# Autodesk Inventor assembly: Cylinder Assembly
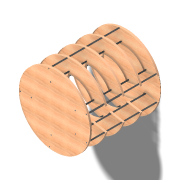
[picture p0: Inventor's stored thumbnail of the model, 180x180]
Saved by Autodesk Inventor 2021 (Build 250183000, 183)
## iProperties
Created: 2020-11-06
Part Number: Cylinder Assembly
Document SubType Name: Assembly
Designer: Dan Wikman
Author: Dan Wikman
## Documents named in this file (12)
- C:\Users\Dan Wikman\OneDrive\University Life\2020, Semester 1\METR4900 Honours Thesis\Cylindrical Mock Up\Cylinder Assembly.iam
- C:\Users\Dan Wikman\OneDrive\University Life\2020, Semester 1\METR4900 Honours Thesis\Cylindrical Mock Up\Rod.ipt
- C:\Users\Dan Wikman\OneDrive\University Life\2020, Semester 1\METR4900 Honours Thesis\Cylindrical Mock Up\Shelf.ipt
- C:\Users\Dan Wikman\OneDrive\University Life\2020, Semester 1\METR4900 Honours Thesis\Cylindrical Mock Up\TopandBase.ipt
- C:\Users\Dan Wikman\OneDrive\University Life\2020, Semester 1\METR4900 Honours Thesis\Cylindrical Mock Up\Shelf Edge Banding.ipt
- C:\Users\Dan Wikman\OneDrive\University Life\2020, Semester 1\METR4900 Honours Thesis\Cylindrical Mock Up\Roof Banding.ipt
- C:\Users\Dan Wikman\OneDrive\University Life\2020, Semester 1\METR4900 Honours Thesis\Cylindrical Mock Up\Cylinder Assembly\AIP\FEA\df0owmtmo.fins
- C:\Users\Dan Wikman\OneDrive\University Life\2020, Semester 1\METR4900 Honours Thesis\Cylindrical Mock Up\Cylinder Assembly\AIP\FEA\df0owmtmo.fsat
- C:\Users\Dan Wikman\OneDrive\University Life\2020, Semester 1\METR4900 Honours Thesis\Cylindrical Mock Up\Cylinder Assembly\AIP\FEA\df0owmtmo.ftes
- C:\Users\Dan Wikman\OneDrive\University Life\2020, Semester 1\METR4900 Honours Thesis\Cylindrical Mock Up\Cylinder Assembly\AIP\FEA\df0owmtmo.fwiz
- C:\Users\Dan Wikman\OneDrive\University Life\2020, Semester 1\METR4900 Honours Thesis\Cylindrical Mock Up\Cylinder Assembly\AIP\FEA\df0owmtq8.fmsh
- C:\Users\Dan Wikman\OneDrive\University Life\2020, Semester 1\METR4900 Honours Thesis\Cylindrical Mock Up\Cylinder Assembly\AIP\FEA\df0owmtq9.fres
## Components (20 placed, 5 different names)
1. Rod:1 — Mate:3, Flush:1, Mate:4, Flush:2
2. Shelf:1 — Mate:1, Mate:2, Mate:3, Mate:26, Mate:27, Flush:7
3. TopandBase:1 — Mate:1, Mate:2, Flush:1, Mate:5, Mate:6, Mate:7, Mate:8, Mate:9, Mate:10, Mate:11, Mate:12, Mate:13, Mate:14, Mate:28, Mate:38, Mate:45, Flush:11
4. TopandBase:2 — Mate:4, Mate:5, Flush:2, Mate:43, Mate:46
5. Rod:2 — Mate:8
6. Rod:3 — Mate:9
7. Rod:4 — Mate:10
8. Rod:5 — Mate:11
9. Rod:6 — Mate:12
10. Rod:7 — Mate:13, Mate:33, Mate:35
11. Rod:8 — Mate:14, Mate:34, Mate:36
12. Rod:9 — Mate:7
13. Rod:10 — Mate:6
14. Shelf Edge Banding:1 — Mate:26, Mate:27, Flush:7, Mate:28
15. Shelf:2 — Mate:33, Mate:34
16. Shelf Edge Banding:2 — Mate:38
17. Shelf:3 — Mate:35, Mate:36
18. Shelf Edge Banding:3 — Flush:10, Mate:44, Mate:46
19. Shelf Edge Banding:4 — Mate:43, Flush:10, Mate:44
20. Roof Banding:1 — Mate:45, Flush:11
## Relationships (37: Mate 30, Flush 7)
- Mate:1: Shelf:1 ↔ TopandBase:1
- Mate:2: Shelf:1 ↔ TopandBase:1
- Mate:3: Rod:1 ↔ Shelf:1
- Flush:1: Rod:1 ↔ TopandBase:1
- Mate:4: Rod:1 ↔ TopandBase:2
- Mate:5: TopandBase:1 ↔ TopandBase:2
- Flush:2: Rod:1 ↔ TopandBase:2
- Mate:6: TopandBase:1 ↔ Rod:10
- Mate:7: TopandBase:1 ↔ Rod:9
- Mate:8: TopandBase:1 ↔ Rod:2
- Mate:9: TopandBase:1 ↔ Rod:3
- Mate:10: TopandBase:1 ↔ Rod:4
- Mate:11: TopandBase:1 ↔ Rod:5
- Mate:12: TopandBase:1 ↔ Rod:6
- Mate:13: TopandBase:1 ↔ Rod:7
- Mate:14: TopandBase:1 ↔ Rod:8
- Mate:26: Shelf:1 ↔ Shelf Edge Banding:1
- Mate:27: Shelf:1 ↔ Shelf Edge Banding:1
- Flush:7 (2 mm): Shelf:1 ↔ Shelf Edge Banding:1
- Mate:28 (274.5 mm): TopandBase:1 ↔ Shelf Edge Banding:1
- [Mate]: Shelf:2 ↔ Shelf Edge Banding:2
- [Mate]: Shelf:2 ↔ Shelf Edge Banding:2
- [Flush] (2 mm): Shelf:2 ↔ Shelf Edge Banding:2
- [Mate]: Shelf:3 ↔ Shelf Edge Banding:3
- [Mate]: Shelf:3 ↔ Shelf Edge Banding:3
- [Flush] (2 mm): Shelf:3 ↔ Shelf Edge Banding:3
- Mate:33: Rod:7 ↔ Shelf:2
- Mate:34: Rod:8 ↔ Shelf:2
- Mate:35: Rod:7 ↔ Shelf:3
- Mate:36: Rod:8 ↔ Shelf:3
- Mate:38 (558 mm): TopandBase:1 ↔ Shelf Edge Banding:2
- Mate:43 (-9 mm): TopandBase:2 ↔ Shelf Edge Banding:4
- Flush:10: Shelf Edge Banding:3 ↔ Shelf Edge Banding:4
- Mate:44: Shelf Edge Banding:3 ↔ Shelf Edge Banding:4
- Mate:45: TopandBase:1 ↔ Roof Banding:1
- Flush:11 (-2 mm): TopandBase:1 ↔ Roof Banding:1
- Mate:46 (274.5 mm): TopandBase:2 ↔ Shelf Edge Banding:3
## Named parameters: sa_0 = 500, d49_d45 = 0 mm, d50_d46 = 0 mm, d51_d47 = 2 mm, d52_d45 = 0 mm, d53_d46 = 0 mm, d54_d47 = 2 mm
note: some values were not read from the file. Shown as the stored number, unit unknown: "sa_0".
